# Autodesk Inventor assembly: Interactive toys a
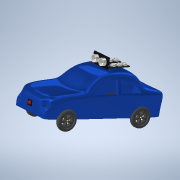
[picture p0: Inventor's stored thumbnail of the model, 180x180]
Saved by Autodesk Inventor 2021 (Build 250183000, 183)
## iProperties
Created: 2021-06-29
Part Number: Interactive toys a
Document SubType Name: Assembly
Designer: Manojgouda K R
Author: Manojgouda K R
## Documents named in this file (7)
- C:\Users\Manojgouda K R\Documents\Auto desk P\IT\Interactive toys a.iam
- C:\Users\Manojgouda K R\Documents\Auto desk P\IT\It 2.iam
- C:\Users\Manojgouda K R\Documents\Auto desk P\IT\Wheel 2.ipt
- C:\Users\Manojgouda K R\Documents\Auto desk P\IT\Base 2.ipt
- C:\Users\Manojgouda K R\Documents\Auto desk P\IT\US sensor.ipt
- C:\Users\Manojgouda K R\Documents\Auto desk P\IT\BUTTON.ipt
- C:\Users\Manojgouda K R\Documents\Auto desk P\IT\button 2.ipt
## Components (16 placed, 6 different names)
1. It 2:1 [sub-assembly] — Mate:1, Mate:2, Flush:1, Flush:2, Mate:3, Flush:3
2. Wheel 2:1 — Mate:1, Mate:2, Flush:7, Mate:16
3. Base 2:1 — Mate:3, Flush:3, Mate:4, 50, Mate:5, Angle:2, Flush:7
4. US sensor:1 — Mate:6
5. BUTTON:1 — Mate:7
6. button 2:1 — Mate:14
7. button 2:2 — Mate:12
8. button 2:3 — Mate:9
9. button 2:4 — Mate:13
10. button 2:5 — Mate:11
11. button 2:6 — Mate:10
12. button 2:7 — Mate:8
13. button 2:8 — Mate:15
14. Wheel 2:2 — Mate:16
15. Wheel 2:3
16. Wheel 2:4
## Relationships (25: Mate 16, Flush 7, Angle 2)
- Mate:1: It 2:1 ↔ Wheel 2:1
- Mate:2: It 2:1 ↔ Wheel 2:1
- Flush:1: It 2:1
- Flush:2: It 2:1
- Mate:3 (0.4 mm): It 2:1 ↔ Base 2:1
- Flush:3: It 2:1 ↔ Base 2:1
- Mate:4: Base 2:1
- 50 [Angle] (37 deg): Base 2:1
- Mate:5: Base 2:1
- Angle:2 (117 deg): Base 2:1
- Flush:4 (-23 mm)
- Flush:5 (-2.75 mm)
- Flush:6 (-2 mm)
- Mate:6: US sensor:1
- Mate:7: BUTTON:1
- Mate:8: button 2:7
- Mate:9: button 2:3
- Mate:10: button 2:6
- Mate:11: button 2:5
- Mate:12: button 2:2
- Mate:13: button 2:4
- Mate:14: button 2:1
- Mate:15: button 2:8
- Flush:7 (0.2 mm): Wheel 2:1 ↔ Base 2:1
- Mate:16 (22 mm): Wheel 2:1 ↔ Wheel 2:2
